# Autodesk Inventor assembly: manifold assembly_MIR2
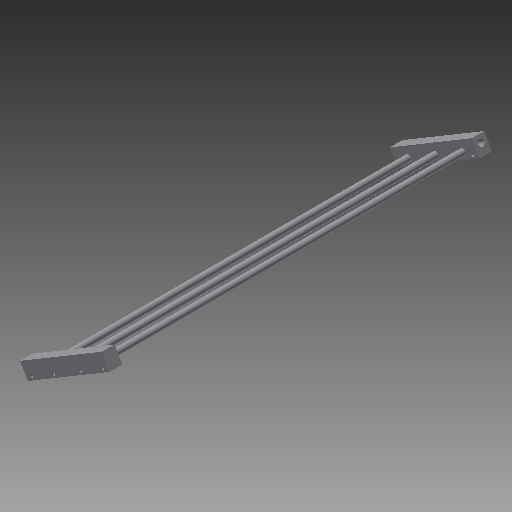
[picture p0: Inventor's stored thumbnail of the model, 512x512]
Saved by Autodesk Inventor 2018 (Build 220112000, 112)
## iProperties
Created: 2018-06-18
Part Number: manifold assembly_MIR2
Document SubType Name: Assembly
Designer: John Viljoen
Author: John Viljoen
## Documents named in this file (3)
- C:\Users\John Viljoen\Documents\Inventor\computer project\manifold assembly_MIR2.iam
- C:\Users\John Viljoen\Documents\Inventor\computer project\manifold mirror_MIR2.ipt
- C:\Users\John Viljoen\Documents\Inventor\computer project\coverplate pipe_MIR2.ipt
## Components (5 placed, 2 different names)
1. manifold mirror_MIR2:1 — Mate:7, Mate:6, Mate:2, Mate:1, Mate:9, Mate:8
2. coverplate pipe_MIR2:1 — Mate:7, Mate:6, Mate:5
3. coverplate pipe_MIR2:2 — Mate:2, Mate:1, Mate:10, Mate:3
4. coverplate pipe_MIR2:3 — Mate:9, Mate:8
5. manifold mirror_MIR2:2 — Mate:10, Mate:5, Mate:3
## Relationships (9: Mate 9)
- Mate:7: manifold mirror_MIR2:1 ↔ coverplate pipe_MIR2:1
- Mate:6 (-0.5 mm): manifold mirror_MIR2:1 ↔ coverplate pipe_MIR2:1
- Mate:2 (-0.5 mm): manifold mirror_MIR2:1 ↔ coverplate pipe_MIR2:2
- Mate:1: manifold mirror_MIR2:1 ↔ coverplate pipe_MIR2:2
- Mate:9 (-0.5 mm): manifold mirror_MIR2:1 ↔ coverplate pipe_MIR2:3
- Mate:8: manifold mirror_MIR2:1 ↔ coverplate pipe_MIR2:3
- Mate:10 (-0.5 mm): coverplate pipe_MIR2:2 ↔ manifold mirror_MIR2:2
- Mate:5: coverplate pipe_MIR2:1 ↔ manifold mirror_MIR2:2
- Mate:3: coverplate pipe_MIR2:2 ↔ manifold mirror_MIR2:2
